# Autodesk Inventor assembly: M90S_ali
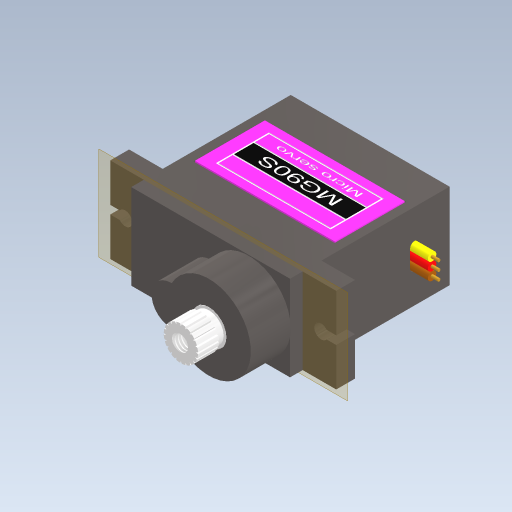
[picture p0: Inventor's stored thumbnail of the model, 512x512]
Saved by Autodesk Inventor 2023.5 (Build 275446000, 446)
## iProperties
Created: 2024-09-01
Part Number: M90S_ali
Description: FreeCAD Model
Document SubType Name: Assembly
Designer: Guntur
Authority: Unknown
Title: Open CASCADE Shape Model
Sending System: FreeCAD
Preprocessor: Open CASCADE STEP processor 7.6
## Documents named in this file (11)
- C:\Users\Guntur\Downloads\mg90s-micro-servo-2.snapshot.3\M90S_ali\M90S_ali.iam
- C:\Users\Guntur\Downloads\mg90s-micro-servo-2.snapshot.3\M90S_ali\axe.ipt
- C:\Users\Guntur\Downloads\mg90s-micro-servo-2.snapshot.3\M90S_ali\base001.ipt
- C:\Users\Guntur\Downloads\mg90s-micro-servo-2.snapshot.3\M90S_ali\etiquette.ipt
- C:\Users\Guntur\Downloads\mg90s-micro-servo-2.snapshot.3\M90S_ali\Tube.ipt
- C:\Users\Guntur\Downloads\mg90s-micro-servo-2.snapshot.3\M90S_ali\Cylindre.ipt
- C:\Users\Guntur\Downloads\mg90s-micro-servo-2.snapshot.3\M90S_ali\Tube001.ipt
- C:\Users\Guntur\Downloads\mg90s-micro-servo-2.snapshot.3\M90S_ali\Tube002.ipt
- C:\Users\Guntur\Downloads\mg90s-micro-servo-2.snapshot.3\M90S_ali\etiquette001.ipt
- C:\Users\Guntur\Downloads\mg90s-micro-servo-2.snapshot.3\M90S_ali\Cylindre001.ipt
- C:\Users\Guntur\Downloads\mg90s-micro-servo-2.snapshot.3\M90S_ali\Cylindre002.ipt
## Components (10 placed, 10 different names)
1. 1
2. 2 — Mate:1, Angle:1
3. 3
4. 4
5. 5
6. 6
7. 7
8. 8
9. 9
10. 10
## Relationships (2: Mate 1, Angle 1)
- Mate:1: 2
- Angle:1 (0 deg): 2
